# Autodesk Inventor assembly: Assembly1
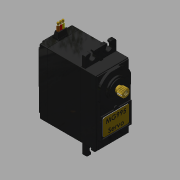
[picture p0: Inventor's stored thumbnail of the model, 180x180]
Saved by Autodesk Inventor 2019 (Build 230136000, 136)
## iProperties
Created: 2021-10-30
Part Number: Assembly1
Document SubType Name: Assembly
Designer: Mohamed
Author: Mohamed
## Documents named in this file (4)
- F:\Semester 7\Design of mechatronics 1\IndustrialLine\SortingAndStorage\Inventor\SSCARA Robot\Assembly1.iam
- F:\Semester 7\Design of mechatronics 1\SSCARA Robot\g_servo body 2.ipt
- F:\Semester 7\Design of mechatronics 1\SSCARA Robot\g_servo mount body.ipt
- F:\Semester 7\Design of mechatronics 1\SSCARA Robot\MG995.ipt
## Components (3 placed, 3 different names)
1. g_servo body 2:1 — Mate:1, Mate:2, Mate:3, Mate:4
2. g_servo mount body:1 — Mate:1, Mate:2, Mate:3, Mate:4, Mate:5, Mate:6
3. MG995:1 — Mate:5, Mate:6
## Relationships (6: Mate 6)
- Mate:1: g_servo body 2:1 ↔ g_servo mount body:1
- Mate:2: g_servo body 2:1 ↔ g_servo mount body:1
- Mate:3: g_servo body 2:1 ↔ g_servo mount body:1
- Mate:4: g_servo body 2:1 ↔ g_servo mount body:1
- Mate:5: g_servo mount body:1 ↔ MG995:1
- Mate:6: g_servo mount body:1 ↔ MG995:1
